# Autodesk Inventor assembly: Frame and Wheels
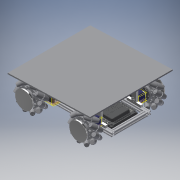
[picture p0: Inventor's stored thumbnail of the model, 180x180]
Saved by Autodesk Inventor 2019 (Build 230136000, 136)
## iProperties
Created: 2019-03-05
Part Number: Frame and Wheels
Document SubType Name: Assembly
Designer: Delta
Mass: 6618.59 g
Surface Area: 22940.3 cm^2
Volume: 3791.34 cm^3
Density: 1.74571 g/cm^3
Author: Delta
## Documents named in this file (9)
- C:\Robotics\CAD\2019-20_CAD\offseason\drive train\Frame and Wheels.iam
- C:\Robotics\CAD\2019-20_CAD\offseason\drive train\Wheel Sub-Assembly.iam
- C:\Robotics\CAD\2019-20_CAD\offseason\drive train\Motor Block.ipt
- C:\Robotics\CAD\COTSParts\Bosch Extrusion\Bosch 20x20 17.5 in.ipt
- C:\Robotics\CAD\COTSParts\Bosch Extrusion\Bosch 20x20 6.75 in.ipt
- C:\Robotics\CAD\2019-20_CAD\offseason\drive train\Top Plate.ipt
- C:\Robotics\CAD\COTSParts\Rev\REV-31-1153RevHub.ipt
- C:\Robotics\CAD\COTSParts\Hinges\1603A230_Hinge.iam
- C:\Robotics\CAD\2019-20_CAD\offseason\drive train\HingeBrace.ipt
## Components (20 placed, 8 different names)
1. Wheel Sub-Assembly:1 [sub-assembly] — Insert:2, Angle:2
2. Wheel Sub-Assembly:2 [sub-assembly] — Insert:4, Angle:4
3. Wheel Sub-Assembly:3 [sub-assembly] — Insert:1, Angle:1
4. Wheel Sub-Assembly:4 [sub-assembly] — Insert:3, Angle:3
5. Motor Block:1 — Insert:1, Mate:1, Flush:1, Mate:2, Angle:1
6. Motor Block:2 — Insert:3, Mate:5, Flush:3, Mate:6, Angle:3
7. Motor Block:3 — Insert:2, Mate:3, Flush:2, Mate:4, Angle:2
8. Motor Block:4 — Mate:7, Flush:4, Mate:8, Insert:4, Angle:4
9. Bosch 20x20 17.5 in:1 — Mate:1, Flush:1, Mate:2, Mate:3, Flush:2, Mate:4, Mate:9, Flush:7, Flush:8, Flush:9, Mate:11, Mate:12, Symmetry:1
10. Bosch 20x20 17.5 in:2 — Mate:5, Flush:3, Mate:6, Mate:7, Flush:4, Mate:8, Flush:5, Flush:6, Mate:10, Flush:10, Flush:11, Symmetry:1
11. Bosch 20x20 6.75 in:1 — Flush:9, Mate:10, Mate:11, Flush:10, Mate:13, Flush:15, Flush:16, Mate:21, Mate:22
12. Bosch 20x20 6.75 in:2 — Flush:5, Flush:6, Mate:9, Flush:7, Flush:8
13. Bosch 20x20 6.75 in:3 — Flush:11, Mate:12, Mate:13
14. Top Plate:1 — Mate:15, Mate:16, Mate:17, Flush:13, Flush:14, Mate:18, Mate:19
15. REV-31-1153RevHub:1
16. REV-31-1153RevHub:2
17. 1603A230_Hinge:1 [sub-assembly] — Mate:16, Flush:13, Mate:19, Flush:15, Insert:5, Insert:6
18. 1603A230_Hinge:2 [sub-assembly] — Mate:17, Flush:14, Mate:18, Flush:16, Insert:7, Insert:8
19. HingeBrace:1 — Mate:22, Insert:5, Insert:6
20. HingeBrace:2 — Mate:21, Insert:7, Insert:8
## Relationships (48: Mate 20, Flush 15, Insert 8, Angle 4, Symmetry 1)
- Insert:1: Wheel Sub-Assembly:3 ↔ Motor Block:1
- Mate:1: Motor Block:1 ↔ Bosch 20x20 17.5 in:1
- Flush:1 (3.65 mm): Motor Block:1 ↔ Bosch 20x20 17.5 in:1
- Mate:2 (-76.2 mm): Motor Block:1 ↔ Bosch 20x20 17.5 in:1
- Insert:2: Wheel Sub-Assembly:1 ↔ Motor Block:3
- Angle:1 (180 deg): Wheel Sub-Assembly:3 ↔ Motor Block:1
- Mate:3: Motor Block:3 ↔ Bosch 20x20 17.5 in:1
- Flush:2 (3.65 mm): Motor Block:3 ↔ Bosch 20x20 17.5 in:1
- Mate:4 (-76.2 mm): Motor Block:3 ↔ Bosch 20x20 17.5 in:1
- Angle:2 (0 deg): Wheel Sub-Assembly:1 ↔ Motor Block:3
- Insert:3: Wheel Sub-Assembly:4 ↔ Motor Block:2
- Mate:5: Motor Block:2 ↔ Bosch 20x20 17.5 in:2
- Flush:3 (-3.65 mm): Motor Block:2 ↔ Bosch 20x20 17.5 in:2
- Mate:6 (-76.2 mm): Motor Block:2 ↔ Bosch 20x20 17.5 in:2
- Angle:3 (0 deg): Wheel Sub-Assembly:4 ↔ Motor Block:2
- Mate:7: Motor Block:4 ↔ Bosch 20x20 17.5 in:2
- Flush:4 (3.65 mm): Motor Block:4 ↔ Bosch 20x20 17.5 in:2
- Mate:8 (-76.2 mm): Motor Block:4 ↔ Bosch 20x20 17.5 in:2
- Insert:4: Wheel Sub-Assembly:2 ↔ Motor Block:4
- Angle:4 (180 deg): Wheel Sub-Assembly:2 ↔ Motor Block:4
- Flush:5: Bosch 20x20 17.5 in:2 ↔ Bosch 20x20 6.75 in:2
- Flush:6: Bosch 20x20 17.5 in:2 ↔ Bosch 20x20 6.75 in:2
- Mate:9: Bosch 20x20 17.5 in:1 ↔ Bosch 20x20 6.75 in:2
- Flush:7: Bosch 20x20 17.5 in:1 ↔ Bosch 20x20 6.75 in:2
- Flush:8: Bosch 20x20 17.5 in:1 ↔ Bosch 20x20 6.75 in:2
- Flush:9: Bosch 20x20 17.5 in:1 ↔ Bosch 20x20 6.75 in:1
- Mate:10: Bosch 20x20 17.5 in:2 ↔ Bosch 20x20 6.75 in:1
- Mate:11: Bosch 20x20 17.5 in:1 ↔ Bosch 20x20 6.75 in:1
- Flush:10: Bosch 20x20 17.5 in:2 ↔ Bosch 20x20 6.75 in:1
- Flush:11: Bosch 20x20 17.5 in:2 ↔ Bosch 20x20 6.75 in:3
- Mate:12: Bosch 20x20 17.5 in:1 ↔ Bosch 20x20 6.75 in:3
- Mate:13 (190.5 mm): Bosch 20x20 6.75 in:1 ↔ Bosch 20x20 6.75 in:3
- Symmetry:1: Bosch 20x20 17.5 in:1 ↔ Bosch 20x20 17.5 in:2
- Mate:15 (-222.25 mm): Top Plate:1
- Mate:16: Top Plate:1 ↔ 1603A230_Hinge:1
- Mate:17: Top Plate:1 ↔ 1603A230_Hinge:2
- Flush:13 (114.3 mm): Top Plate:1 ↔ 1603A230_Hinge:1
- Flush:14 (-114.3 mm): Top Plate:1 ↔ 1603A230_Hinge:2
- Mate:18 (-12.7 mm): Top Plate:1 ↔ 1603A230_Hinge:2
- Mate:19 (-12.7 mm): Top Plate:1 ↔ 1603A230_Hinge:1
- Flush:15: Bosch 20x20 6.75 in:1 ↔ 1603A230_Hinge:1
- Flush:16: Bosch 20x20 6.75 in:1 ↔ 1603A230_Hinge:2
- Mate:21: Bosch 20x20 6.75 in:1 ↔ HingeBrace:2
- Mate:22: Bosch 20x20 6.75 in:1 ↔ HingeBrace:1
- Insert:5: 1603A230_Hinge:1 ↔ HingeBrace:1
- Insert:6: 1603A230_Hinge:1 ↔ HingeBrace:1
- Insert:7: 1603A230_Hinge:2 ↔ HingeBrace:2
- Insert:8: 1603A230_Hinge:2 ↔ HingeBrace:2
